# Autodesk Inventor assembly: Motor
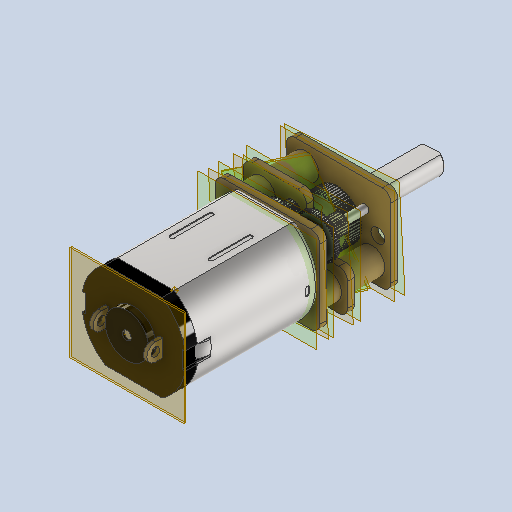
[picture p0: Inventor's stored thumbnail of the model, 512x512]
Saved by Autodesk Inventor 2023 (Build 270158000, 158)
## iProperties
Created: 2021-01-29
Part Number: Motor
Document SubType Name: Assembly
Designer: João
Author: João
## Documents named in this file (24)
- G:\My Drive\CAD File Sharing\Inventor\Birty\Motors\Motor.iam
- G:\My Drive\CAD File Sharing\Inventor\Birty\Motors\Base.ipt
- G:\My Drive\CAD File Sharing\Inventor\Birty\Motors\Rotor.ipt
- G:\My Drive\CAD File Sharing\Inventor\Birty\Motors\Carcaça.ipt
- G:\My Drive\CAD File Sharing\Inventor\Birty\Motors\Apoio Contato.ipt
- G:\My Drive\CAD File Sharing\Inventor\Birty\Motors\Contato.ipt
- G:\My Drive\CAD File Sharing\Inventor\Birty\Motors\Suporte Contato.ipt
- G:\My Drive\CAD File Sharing\Inventor\Birty\Motors\Suporte Bobinas.ipt
- G:\My Drive\CAD File Sharing\Inventor\Birty\Motors\Imãs.ipt
- G:\My Drive\CAD File Sharing\Inventor\Birty\Motors\Terminais.ipt
- G:\My Drive\CAD File Sharing\Inventor\Birty\Motors\Chapa Inferior.ipt
- G:\My Drive\CAD File Sharing\Inventor\Birty\Motors\Escovas.ipt
- G:\My Drive\CAD File Sharing\Inventor\Birty\Motors\Chapa Intermediária.ipt
- G:\My Drive\CAD File Sharing\Inventor\Birty\Motors\Chapa Superior.ipt
- G:\My Drive\CAD File Sharing\Inventor\Birty\Motors\Eixo Maior - Engrenagem.ipt
- G:\My Drive\CAD File Sharing\Inventor\Birty\Motors\Eixo Médio - Engrenagem.ipt
- G:\My Drive\CAD File Sharing\Inventor\Birty\Motors\Parafuso.ipt
- G:\My Drive\CAD File Sharing\Inventor\Birty\Motors\Eixo Menor - Engrenagem.ipt
- M:\Autodesk\Inventor 2023\Common Models\N20 Motors\GearMotor\Montagem1\Design Accelerator\Engrenagens retas2.iam
- M:\Autodesk\Inventor 2023\Common Models\N20 Motors\GearMotor\Montagem1\Design Accelerator\Engrenagens retas1.iam
- G:\My Drive\CAD File Sharing\Inventor\Birty\Motors\Eixo - Encaixe D.ipt
- M:\Autodesk\Inventor 2023\Common Models\N20 Motors\GearMotor\Montagem1\Design Accelerator\Engrenagens retas5.iam
- M:\Autodesk\Inventor 2023\Common Models\N20 Motors\GearMotor\Montagem1\Design Accelerator\Engrenagens retas7.iam
- M:\Autodesk\Inventor 2023\Common Models\N20 Motors\GearMotor\Montagem1\Design Accelerator\Engrenagens retas8.iam
## Components (25 placed, 19 different names)
1. Base:1 — Coincidente:1, Coincidente:15, Coincidente:18, Coincidente:20, Ângulo:1, Coincidente:21, Ângulo:2, Alinhado:2, Coincidente:26, Ângulo:3, Alinhado:13, Coincidente:75, Coincidente:76, Coincidente:80
2. Rotor:1 — Coincidente:1, Coincidente:7, Coincidente:9, Coincidente:24, Coincidente:27, Coincidente:32, Coincidente:33, Coincidente:43, Alinhado:14, Coincidente:46, Rotação:1
3. Apoio Contato:1 — Coincidente:7, Coincidente:10
4. Contato:1 — Coincidente:8, Coincidente:10, Coincidente:11, Ângulo:4, Rotação:12
5. Suporte Contato:1 — Coincidente:8, Coincidente:9, Coincidente:11, Ângulo:4, Coincidente:44, Coincidente:83, Rotação:12
6. Imãs:1 — Coincidente:32, Alinhado:4, Tangente:1
7. Terminais:1 — Coincidente:20, Ângulo:1, Coincidente:23
8. Terminais:2 — Coincidente:21, Ângulo:2, Coincidente:22, Coincidente:26, Coincidente:30
9. Escovas:1 — Coincidente:27, Ângulo:3, Coincidente:28, Coincidente:29
10. Chapa Inferior:1 — Coincidente:24, Coincidente:34, Ângulo:6, Ângulo:7, Coincidente:37, Alinhado:10, Alinhado:12, Coincidente:81, Ângulo:8
11. Chapa Intermediária:1 — Coincidente:33, Coincidente:34, Ângulo:6, Coincidente:35, Coincidente:36, Coincidente:39, Coincidente:45, Alinhado:16, Alinhado:17, Coincidente:55, Rotação:11
12. Chapa Superior:1 — Coincidente:35, Coincidente:36, Ângulo:7, Alinhado:6, Coincidente:41, Coincidente:42, Alinhado:7, Alinhado:8, Coincidente:54, Alinhado:20, Rotação:7, Rotação:8, Rotação:9, Rotação:10
13. Eixo Maior - Engrenagem:1 — Coincidente:37, Coincidente:38, Coincidente:52, Coincidente:63, Rotação:9
14. Eixo Médio - Engrenagem:1 — Coincidente:39, Coincidente:40, Coincidente:69, Coincidente:70, Rotação:10
15. Parafuso:1 — Coincidente:41, Alinhado:7, Rotação:7
16. Parafuso:2 — Coincidente:42, Alinhado:8, Rotação:8
17. Suporte Bobinas:2 — Coincidente:43, Coincidente:44, Alinhado:9, Coincidente:83
18. Eixo Menor - Engrenagem:1 — Coincidente:45, Alinhado:11, Coincidente:48, Coincidente:50, Rotação:11
19. Engrenagens retas:1 [sub-assembly] — Coincidente:46, Coincidente:47, Coincidente:48, Coincidente:49, Alinhado:15, Rotação:1, Rotação:2
20. Engrenagens retas:2 [sub-assembly] — Coincidente:50, Coincidente:51, Coincidente:52, Coincidente:53, Coincidente:64, Rotação:2, Rotação:3
21. Eixo - Encaixe D:1 — Coincidente:54, Coincidente:55, Coincidente:65, Coincidente:67, Coincidente:72, Rotação:6
22. Engrenagens retas:3 [sub-assembly] — Coincidente:63, Coincidente:64, Coincidente:65, Coincidente:66, Coincidente:68, Coincidente:82, Rotação:3, Rotação:4
23. Engrenagens retas:4 [sub-assembly] — Alinhado:18, Coincidente:67, Coincidente:68, Coincidente:69, Alinhado:19, Alinhado:21, Coincidente:82, Rotação:4, Rotação:5
24. Engrenagens retas:5 [sub-assembly] — Coincidente:70, Coincidente:71, Coincidente:72, Coincidente:73, Rotação:5, Rotação:6
25. Carcaça:1 — Coincidente:74, Coincidente:77, Coincidente:80, Coincidente:81, Ângulo:8, Tangente:1
## Relationships (102: Mate 64, Flush 18, RelateRotation 12, Angle 7, Tangent 1)
- Coincidente:1 [Mate]: Base:1 ↔ Rotor:1
- Coincidente:7 [Mate]: Rotor:1 ↔ Apoio Contato:1
- Coincidente:8 [Mate]: Contato:1 ↔ Suporte Contato:1
- Coincidente:9 [Mate]: Rotor:1 ↔ Suporte Contato:1
- Coincidente:10 [Mate]: Apoio Contato:1 ↔ Contato:1
- Coincidente:11 [Mate]: Contato:1 ↔ Suporte Contato:1
- Coincidente:15 [Mate]: Base:1
- Coincidente:18 [Mate]: Base:1
- Coincidente:19 [Mate]
- Coincidente:20 [Mate]: Base:1 ↔ Terminais:1
- Ângulo:1 [Angle] (0 deg): Base:1 ↔ Terminais:1
- Coincidente:21 [Mate]: Base:1 ↔ Terminais:2
- Ângulo:2 [Angle] (0 deg): Base:1 ↔ Terminais:2
- Coincidente:22 [Mate]: Terminais:2
- Coincidente:23 [Mate]: Terminais:1
- Coincidente:24 [Mate]: Rotor:1 ↔ Chapa Inferior:1
- Alinhado:2 [Flush]: Base:1
- Coincidente:26 [Mate]: Base:1 ↔ Terminais:2
- Coincidente:27 [Mate]: Rotor:1 ↔ Escovas:1
- Ângulo:3 [Angle] (0 deg): Base:1 ↔ Escovas:1
- Coincidente:28 [Mate]: Escovas:1
- Coincidente:29 [Mate]: Escovas:1
- Coincidente:30 [Mate]: Terminais:2
- Ângulo:4 [Angle] (0 deg): Contato:1 ↔ Suporte Contato:1
- Coincidente:32 [Mate]: Rotor:1 ↔ Imãs:1
- Alinhado:4 [Flush]: Imãs:1
- Coincidente:33 [Mate]: Rotor:1 ↔ Chapa Intermediária:1
- Coincidente:34 [Mate]: Chapa Inferior:1 ↔ Chapa Intermediária:1
- Ângulo:6 [Angle] (0 deg): Chapa Inferior:1 ↔ Chapa Intermediária:1
- Coincidente:35 [Mate]: Chapa Intermediária:1 ↔ Chapa Superior:1
- Coincidente:36 [Mate]: Chapa Intermediária:1 ↔ Chapa Superior:1
- Ângulo:7 [Angle] (0 deg): Chapa Inferior:1 ↔ Chapa Superior:1
- Alinhado:6 [Flush] (-0.1 mm): Chapa Superior:1
- Coincidente:37 [Mate]: Chapa Inferior:1 ↔ Eixo Maior - Engrenagem:1
- Coincidente:38 [Mate]: Eixo Maior - Engrenagem:1
- Coincidente:39 [Mate]: Chapa Intermediária:1 ↔ Eixo Médio - Engrenagem:1
- Coincidente:40 [Mate]: Eixo Médio - Engrenagem:1
- Coincidente:41 [Mate]: Chapa Superior:1 ↔ Parafuso:1
- Coincidente:42 [Mate]: Chapa Superior:1 ↔ Parafuso:2
- Alinhado:7 [Flush]: Chapa Superior:1 ↔ Parafuso:1
- Alinhado:8 [Flush]: Chapa Superior:1 ↔ Parafuso:2
- Coincidente:43 [Mate]: Rotor:1 ↔ Suporte Bobinas:2
- Coincidente:44 [Mate]: Suporte Contato:1 ↔ Suporte Bobinas:2
- Alinhado:9 [Flush]: Suporte Bobinas:2
- Coincidente:45 [Mate]: Chapa Intermediária:1 ↔ Eixo Menor - Engrenagem:1
- Alinhado:10 [Flush] (-0.1 mm): Chapa Inferior:1
- Alinhado:11 [Flush]: Eixo Menor - Engrenagem:1
- Alinhado:12 [Flush] (0.15 mm): Chapa Inferior:1
- Alinhado:13 [Flush] (-0.2 mm): Base:1
- Alinhado:14 [Flush]: Rotor:1
- Coincidente:46 [Mate]: Rotor:1 ↔ Engrenagens retas:1
- Coincidente:47 [Mate]: Engrenagens retas:1
- Coincidente:48 [Mate]: Eixo Menor - Engrenagem:1 ↔ Engrenagens retas:1
- Coincidente:49 [Mate]: Engrenagens retas:1
- Alinhado:15 [Flush]: Engrenagens retas:1
- Alinhado:16 [Flush] (0.25 mm): Chapa Intermediária:1
- Coincidente:50 [Mate]: Eixo Menor - Engrenagem:1 ↔ Engrenagens retas:2
- Coincidente:51 [Mate]: Engrenagens retas:2
- Coincidente:52 [Mate]: Eixo Maior - Engrenagem:1 ↔ Engrenagens retas:2
- Coincidente:53 [Mate]: Engrenagens retas:2
- Alinhado:17 [Flush] (0.15 mm): Chapa Intermediária:1
- Coincidente:54 [Mate]: Chapa Superior:1 ↔ Eixo - Encaixe D:1
- Coincidente:55 [Mate]: Chapa Intermediária:1 ↔ Eixo - Encaixe D:1
- Coincidente:63 [Mate]: Eixo Maior - Engrenagem:1 ↔ Engrenagens retas:3
- Coincidente:64 [Mate]: Engrenagens retas:2 ↔ Engrenagens retas:3
- Coincidente:65 [Mate]: Eixo - Encaixe D:1 ↔ Engrenagens retas:3
- Coincidente:66 [Mate]: Engrenagens retas:3
- Alinhado:18 [Flush]: Engrenagens retas:4
- Coincidente:67 [Mate]: Eixo - Encaixe D:1 ↔ Engrenagens retas:4
- Coincidente:68 [Mate]: Engrenagens retas:3 ↔ Engrenagens retas:4
- Coincidente:69 [Mate]: Eixo Médio - Engrenagem:1 ↔ Engrenagens retas:4
- Alinhado:19 [Flush]: Engrenagens retas:4
- Alinhado:20 [Flush] (0.15 mm): Chapa Superior:1
- Alinhado:21 [Flush] (0.1 mm): Engrenagens retas:4
- Coincidente:70 [Mate]: Eixo Médio - Engrenagem:1 ↔ Engrenagens retas:5
- Coincidente:71 [Mate]: Engrenagens retas:5
- Coincidente:72 [Mate]: Eixo - Encaixe D:1 ↔ Engrenagens retas:5
- Coincidente:73 [Mate]: Engrenagens retas:5
- Coincidente:74 [Mate]: Carcaça:1
- Coincidente:75 [Mate]: Base:1
- Coincidente:76 [Mate]: Base:1
- Coincidente:77 [Mate]: Carcaça:1
- Coincidente:78 [Mate]
- Coincidente:79 [Mate]
- Coincidente:80 [Mate]: Base:1 ↔ Carcaça:1
- Coincidente:81 [Mate]: Chapa Inferior:1 ↔ Carcaça:1
- Ângulo:8 [Angle] (0 deg): Chapa Inferior:1 ↔ Carcaça:1
- Coincidente:82 [Mate]: Engrenagens retas:3 ↔ Engrenagens retas:4
- Rotação:1 [RelateRotation] (1 ul): Rotor:1 ↔ Engrenagens retas:1
- Rotação:2 [RelateRotation] (1 ul): Engrenagens retas:1 ↔ Engrenagens retas:2
- Rotação:3 [RelateRotation] (1 ul): Engrenagens retas:2 ↔ Engrenagens retas:3
- Rotação:4 [RelateRotation] (1 ul): Engrenagens retas:3 ↔ Engrenagens retas:4
- Rotação:5 [RelateRotation] (1 ul): Engrenagens retas:4 ↔ Engrenagens retas:5
- Rotação:6 [RelateRotation] (1 ul): Eixo - Encaixe D:1 ↔ Engrenagens retas:5
- Rotação:7 [RelateRotation] (1 ul): Chapa Superior:1 ↔ Parafuso:1
- Rotação:8 [RelateRotation] (1 ul): Chapa Superior:1 ↔ Parafuso:2
- Rotação:9 [RelateRotation] (1 ul): Chapa Superior:1 ↔ Eixo Maior - Engrenagem:1
- Rotação:10 [RelateRotation] (1 ul): Chapa Superior:1 ↔ Eixo Médio - Engrenagem:1
- Rotação:11 [RelateRotation] (1 ul): Chapa Intermediária:1 ↔ Eixo Menor - Engrenagem:1
- Tangente:1: Imãs:1 ↔ Carcaça:1
- Coincidente:83 [Mate]: Suporte Contato:1 ↔ Suporte Bobinas:2
- Rotação:12 [RelateRotation] (1 ul): Contato:1 ↔ Suporte Contato:1
